# Autodesk Inventor assembly: Shift_Shaft
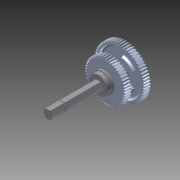
[picture p0: Inventor's stored thumbnail of the model, 180x180]
Saved by Autodesk Inventor 2014 (Build 180170000, 170)
## iProperties
Created: 2014-01-14
Part Number: Shift_Shaft
Document SubType Name: Assembly
Designer: 3D Printer
Author: 3D Printer
## Documents named in this file (9)
- E:\Robotics\Robotics 13-14\Team_0334(Chassis)\Team_334_Dual_Speed\Shift_Shaft.iam
- E:\Robotics\Robotics 13-14\Team_0334(Chassis)\Team_334_Dual_Speed\Shift_Shaft.ipt
- E:\Robotics\Robotics 13-14\Team_0334(Chassis)\Team_334_Dual_Speed\FR8ZZ_Bearing_1.ipt
- E:\Robotics\Robotics 13-14\Team_0334(Chassis)\Team_334_Dual_Speed\48_tooth_dog.ipt
- E:\Robotics\Robotics 13-14\Team_0334(Chassis)\Team_334_Dual_Speed\R8_Bearing.ipt
- E:\Robotics\Robotics 13-14\Team_0334(Chassis)\Team_334_Dual_Speed\60_tooth_dog.ipt
- E:\Robotics\Robotics 13-14\Team_0334(Chassis)\Team_334_Dual_Speed\FR8ZZ-Hex_Bearing.ipt
- E:\Robotics\Robotics 13-14\Team_0334(Chassis)\Team_334_Dual_Speed\Retaining_Ring.ipt
- E:\Robotics\Robotics 13-14\Team_0334(Chassis)\Team_334_Dual_Speed\Spacer.ipt
## Components (10 placed, 8 different names)
1. Shift_Shaft:1 — Insert:1
2. FR8ZZ_Bearing_1:1
3. 48_tooth_dog:1
4. R8_Bearing:1
5. 60_tooth_dog:1
6. FR8ZZ-Hex_Bearing:1
7. Retaining_Ring:1
8. FR8ZZ-Hex_Bearing:2
9. Retaining_Ring:2 — Insert:1
10. Spacer:1
## Relationships (1: Insert 1)
- Insert:1: Shift_Shaft:1 ↔ Retaining_Ring:2
